# Autodesk Inventor assembly: Modul
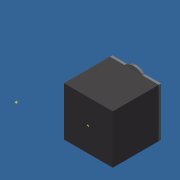
[picture p0: Inventor's stored thumbnail of the model, 180x180]
Saved by Autodesk Inventor 2018.2 (Build 222227000, 227)
## iProperties
Company: Fraunhofer ILT
Created: 2018-10-15
Part Number: Modul
Material: geeigneten Werkstoff auswählen !
Document SubType Name: Assembly
Designer: N.Grubert
Title: =Description
Author: N.Grubert
## Documents named in this file (5)
- C:\Users\GRUBERT\Documents\COSIMA-Laserstar\CAD\Modul.iam
- C:\Users\GRUBERT\Documents\COSIMA-Laserstar\CAD\Modul Deckel.ipt
- C:\Users\GRUBERT\Documents\COSIMA-Laserstar\CAD\Modul Gehäuse.ipt
- C:\Users\GRUBERT\Documents\COSIMA-Laserstar\CAD\SlavesSammelplatine.iam
- C:\Users\GRUBERT\Documents\COSIMA-Laserstar\CAD\Photodiodendummie.ipt
## Components (4 placed, 4 different names)
1. Modul Deckel:1 — Passend:1, Fluchtend:1, Fluchtend:2
2. Modul Gehäuse:1 — Passend:1, Fluchtend:1, Fluchtend:2, Passend:2, Passend:3, Passend:4, Passend:5, Passend:6, Passend:7
3. SlavesSammelplatine:1 [sub-assembly] — Passend:5, Passend:6, Passend:7
4. Photodiodendummie:1
## Relationships (9: Mate 7, Flush 2)
- Passend:1 [Mate]: Modul Deckel:1 ↔ Modul Gehäuse:1
- Fluchtend:1 [Flush]: Modul Deckel:1 ↔ Modul Gehäuse:1
- Fluchtend:2 [Flush]: Modul Deckel:1 ↔ Modul Gehäuse:1
- Passend:2 [Mate]: Modul Gehäuse:1
- Passend:3 [Mate]: Modul Gehäuse:1
- Passend:4 [Mate]: Modul Gehäuse:1
- Passend:5 [Mate] (5 mm): Modul Gehäuse:1 ↔ SlavesSammelplatine:1
- Passend:6 [Mate] (16.25 mm): Modul Gehäuse:1 ↔ SlavesSammelplatine:1
- Passend:7 [Mate]: Modul Gehäuse:1 ↔ SlavesSammelplatine:1
